# Autodesk Inventor assembly: akkufach_2
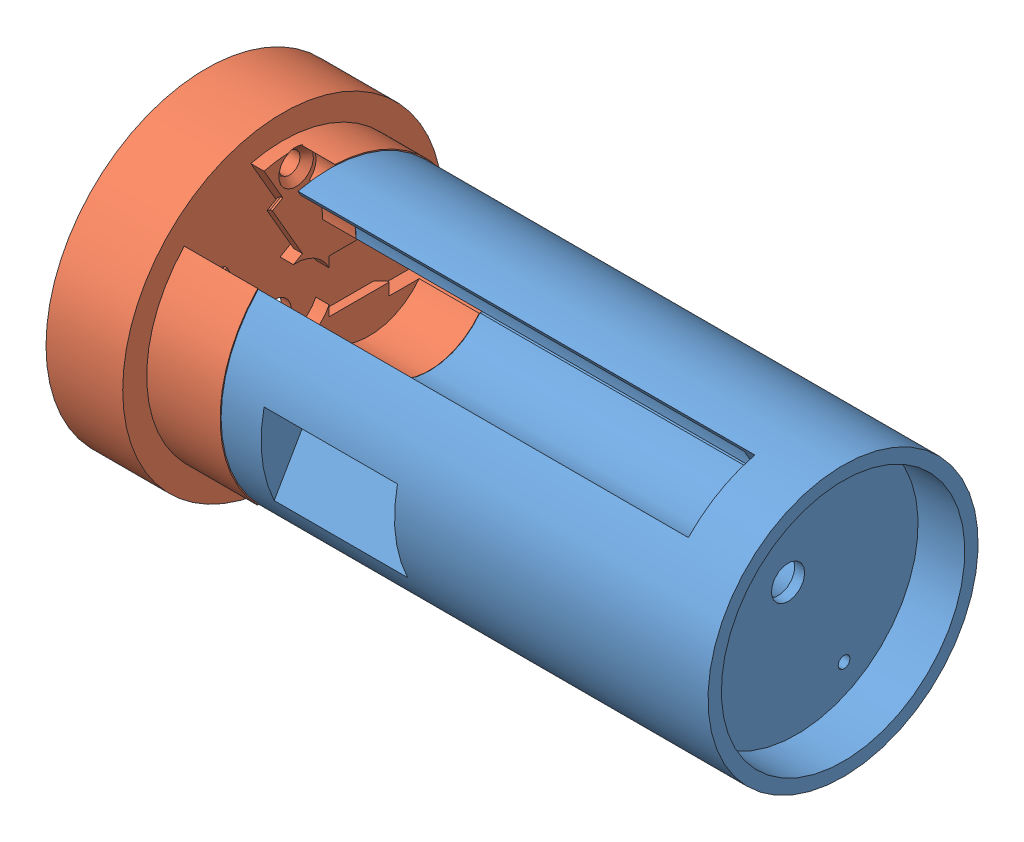
[picture p0: shaded view drawn from the shape stored in the file]
Saved by Autodesk Inventor 2022 (Build 260153000, 153)
## iProperties
Created: 2022-11-02
Part Number: akkufach_2
Document SubType Name: Assembly
Designer: g.schardt
Author: g.schardt
## Documents named in this file (3)
- S:\g.schardt\Inventor\Tauchlampe\batteriefach_komplett.iam
- S:\g.schardt\Inventor\Tauchlampe\batteriefach_deckel.ipt
- S:\g.schardt\Inventor\Tauchlampe\batteriefach.ipt
## Components (2 placed, 2 different names)
1. batteriefach_deckel:1 — Passend:1, Passend:2, Passend:3
2. batteriefach:1 — Passend:1, Passend:2, Passend:3
## Relationships (3: Mate 3)
- Passend:1 [Mate]: batteriefach_deckel:1 ↔ batteriefach:1
- Passend:2 [Mate]: batteriefach_deckel:1 ↔ batteriefach:1
- Passend:3 [Mate]: batteriefach_deckel:1 ↔ batteriefach:1
